# Autodesk Inventor assembly: AM14U3 Long
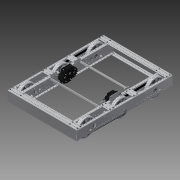
[picture p0: Inventor's stored thumbnail of the model, 180x180]
Saved by Autodesk Inventor 2018 (Build 220112000, 112)
## iProperties
Category: Drive Base
Company: Autodesk Inc.
Created: 2017-12-15
Part Number: AM14U3 Long
Document SubType Name: Assembly
Designer: Autodesk Inc.
Catalog Web Link: http://www.andymark.com/AM14U3-p/am-14u3.htm
Vendor: Andy Mark Inc.
Author: Autodesk Inc.
Keywords: Drive Base Long
## Documents named in this file (2)
- D:\FIRST 2018\FIRST 2018 Inventor\FIRST 2017 Drive Base\DB_DriveBaseLong_AM14U3.iam
- D:\FIRST 2018\FIRST 2018 Inventor\FIRST 2017 Drive Base\Parts\AM14U3 Long Half.iam
## Components (2 placed, 2 different names)
1. AM14U3 Long Half_1 [sub-assembly] — Insert:1, Insert:2, Mate:1
2. AM14U3 Long Half_2 [sub-assembly] — Insert:1, Insert:2
## Relationships (3: Insert 2, Mate 1)
- Insert:1: AM14U3 Long Half_1 ↔ AM14U3 Long Half_2
- Insert:2: AM14U3 Long Half_1 ↔ AM14U3 Long Half_2
- Mate:1: AM14U3 Long Half_1
